# Autodesk Inventor assembly: EvelTallBeam
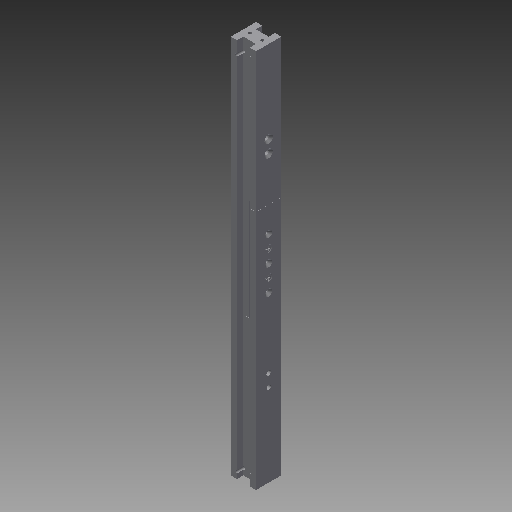
[picture p0: Inventor's stored thumbnail of the model, 512x512]
Saved by Autodesk Inventor 2019 (Build 230136000, 136)
## iProperties
Created: 2019-10-01
Part Number: EvelTallBeam
Document SubType Name: Assembly
Designer: james
Author: james
## Documents named in this file (3)
- F:\JimsDesign\Jims2020FTC\EvelTallBeam.iam
- F:\JimsDesign\Jims2020FTC\TallBeamSplit.ipt
- F:\JimsDesign\Library\McMaster\Screws\91771A152_18-8 SS FLAT HEAD PHILLIPS MACHINE SCREW.ipt
## Components (7 placed, 2 different names)
1. TallBeamSplit:1 — Mate:1, Mate:2, Mate:3, Mate:4, Mate:5, Mate:6, Flush:3, Flush:4, Flush:5
2. TallBeamSplit:2 — Mate:1, Mate:2, Mate:3, Mate:7, Mate:8, Flush:1, Flush:2
3. 91771A152_18-8 SS FLAT HEAD PHILLIPS MACHINE SCREW:1 — Mate:4, Flush:3
4. 91771A152_18-8 SS FLAT HEAD PHILLIPS MACHINE SCREW:2 — Mate:5, Flush:4
5. 91771A152_18-8 SS FLAT HEAD PHILLIPS MACHINE SCREW:3 — Mate:6, Flush:5
6. 91771A152_18-8 SS FLAT HEAD PHILLIPS MACHINE SCREW:4 — Mate:7, Flush:1
7. 91771A152_18-8 SS FLAT HEAD PHILLIPS MACHINE SCREW:5 — Mate:8, Flush:2
## Relationships (13: Mate 8, Flush 5)
- Mate:1: TallBeamSplit:1 ↔ TallBeamSplit:2
- Mate:2: TallBeamSplit:1 ↔ TallBeamSplit:2
- Mate:3: TallBeamSplit:1 ↔ TallBeamSplit:2
- Mate:4: TallBeamSplit:1 ↔ 91771A152_18-8 SS FLAT HEAD PHILLIPS MACHINE SCREW:1
- Mate:5: TallBeamSplit:1 ↔ 91771A152_18-8 SS FLAT HEAD PHILLIPS MACHINE SCREW:2
- Mate:6: TallBeamSplit:1 ↔ 91771A152_18-8 SS FLAT HEAD PHILLIPS MACHINE SCREW:3
- Mate:7: TallBeamSplit:2 ↔ 91771A152_18-8 SS FLAT HEAD PHILLIPS MACHINE SCREW:4
- Mate:8: TallBeamSplit:2 ↔ 91771A152_18-8 SS FLAT HEAD PHILLIPS MACHINE SCREW:5
- Flush:1: TallBeamSplit:2 ↔ 91771A152_18-8 SS FLAT HEAD PHILLIPS MACHINE SCREW:4
- Flush:2: TallBeamSplit:2 ↔ 91771A152_18-8 SS FLAT HEAD PHILLIPS MACHINE SCREW:5
- Flush:3: TallBeamSplit:1 ↔ 91771A152_18-8 SS FLAT HEAD PHILLIPS MACHINE SCREW:1
- Flush:4: TallBeamSplit:1 ↔ 91771A152_18-8 SS FLAT HEAD PHILLIPS MACHINE SCREW:2
- Flush:5: TallBeamSplit:1 ↔ 91771A152_18-8 SS FLAT HEAD PHILLIPS MACHINE SCREW:3
